# Autodesk Inventor assembly: Bullet_v5_SiliconeSample_Assembly
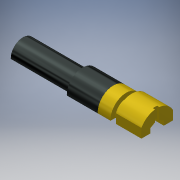
[picture p0: Inventor's stored thumbnail of the model, 180x180]
Saved by Autodesk Inventor 2018 (Build 220112000, 112)
## iProperties
Created: 2018-05-23
Part Number: Bullet_v5_SiliconeSample_Assembly
Document SubType Name: Assembly
Designer: Sergey
Author: Sergey
## Documents named in this file (3)
- D:\Dell_DiskC_Samsung\Documents\Inventor\FlowCryostat17\Bullets\Bullet_v5_Thread\Bullet_v5_SiliconeSample_Assembly.iam
- D:\Dell_DiskC_Samsung\Documents\Inventor\FlowCryostat17\Bullets\Bullet_v5_Thread\Bullet_v5_SiliconeSample.ipt
- D:\Dell_DiskC_Samsung\Documents\Inventor\FlowCryostat17\Bullets\Bullet_v5_Thread\Bullet_v5_SiliconeSample_TopPart.ipt
## Components (2 placed, 2 different names)
1. Bullet_v5_SiliconeSample:1 — Mate:1, Mate:2
2. Bullet_v5_SiliconeSample_TopPart:1 — Mate:1, Mate:2
## Relationships (2: Mate 2)
- Mate:1 (0.0254 mm): Bullet_v5_SiliconeSample:1 ↔ Bullet_v5_SiliconeSample_TopPart:1
- Mate:2: Bullet_v5_SiliconeSample:1 ↔ Bullet_v5_SiliconeSample_TopPart:1
